# Autodesk Inventor assembly: am-3072aDART12
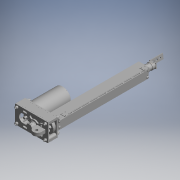
[picture p0: Inventor's stored thumbnail of the model, 180x180]
Saved by Autodesk Inventor 2017 (Build 210142000, 142)
## iProperties
Created: 2016-01-05
Part Number: am-3072aDART12
Description: STEP AP203
Document SubType Name: Assembly
Designer: steele
Sending System: SolidWorks 2014
Preprocessor: SwSTEP 2.0
Title: am-3072a DART 12.STEP
Revision Number: ANY
## Documents named in this file (4)
- C:\snobotics\CAD-Development\robSteele\SnoBotics2016\DART 12inch from AM\am-3072aDART12.iam
- C:\snobotics\CAD-Development\robSteele\SnoBotics2016\DART 12inch from AM\DART Motor Module.iam
- C:\snobotics\CAD-Development\robSteele\SnoBotics2016\DART 12inch from AM\DART 12 Lead Screw Module.iam
- C:\snobotics\CAD-Development\robSteele\SnoBotics2016\2016-05-05-ShooterPrototype\simpleBracketForTopOfDart.ipt
## Components (3 placed, 3 different names)
1. DART Motor Module_1 [sub-assembly]
2. DART 12 Lead Screw Module_2 [sub-assembly] — Insert:1, Flush:1, Flush:2
3. simpleBracketForTopOfDart:1 — Insert:1, Flush:1, Flush:2
## Relationships (3: Flush 2, Insert 1)
- Insert:1: DART 12 Lead Screw Module_2 ↔ simpleBracketForTopOfDart:1
- Flush:1: DART 12 Lead Screw Module_2 ↔ simpleBracketForTopOfDart:1
- Flush:2: DART 12 Lead Screw Module_2 ↔ simpleBracketForTopOfDart:1
